# Autodesk Inventor assembly: main room, doors, corridor connected
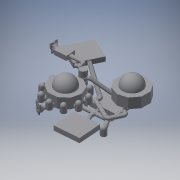
[picture p0: Inventor's stored thumbnail of the model, 180x180]
Saved by Autodesk Inventor 2017 (Build 210142000, 142)
## iProperties
Created: 2018-03-04
Part Number: main room, doors, corridor connected
Document SubType Name: Assembly
Designer: Braxton
Author: Braxton
## Documents named in this file (21)
- E:\School\Game develpment\geoscape\done solid\map\main room, doors, corridor connected.iam
- E:\School\Game develpment\geoscape\done solid\rooms\assembly\main room with double door.iam
- E:\School\Game develpment\geoscape\done solid\corridors\corridor.ipt
- E:\School\Game develpment\geoscape\done solid\corridors\corridor turn.ipt
- E:\School\Game develpment\geoscape\done solid\corridors\Y corridor.ipt
- E:\School\Game develpment\geoscape\done solid\corridors\end cap.ipt
- E:\School\Game develpment\geoscape\done solid\corridors\ramp top connect.ipt
- E:\School\Game develpment\geoscape\done solid\corridors\ramp.ipt
- E:\School\Game develpment\geoscape\done solid\corridors\ramp bottom connect.ipt
- E:\School\Game develpment\geoscape\done solid\corridors\curve ramp.ipt
- E:\School\Game develpment\geoscape\done solid\rooms\assembly\dome with double door.iam
- E:\School\Game develpment\geoscape\done solid\corridors\X corridor.ipt
- E:\School\Game develpment\geoscape\done solid\rooms\room with 15 cubicals.ipt
- E:\School\Game develpment\geoscape\done solid\corridors\ramp connect both ends.ipt
- E:\School\Game develpment\geoscape\done solid\doors\end door\9 foot door\end door room (9).ipt
- E:\School\Game develpment\geoscape\done solid\doors\end door\9 foot door\end door assembly (9).ipt.iam
- E:\School\Game develpment\geoscape\done solid\rooms\assembly\dome one terminal.iam
- E:\School\Game develpment\geoscape\done solid\rooms\assembly\assembly of dome with corridors with all doors.iam
- E:\School\Game develpment\geoscape\doors\end door assembly (closed) (9).ipt.iam
- end door assembly (9).ipt
- end door assembly (closed) (9).ipt
## Components (69 placed, 19 different names)
1. ramp top connect:3 — Flush:84, Insert:77, Flush:103, Insert:87
2. ramp:8 — Insert:74, Flush:81, Insert:75, Flush:82
3. ramp:7 — Insert:75, Flush:82, Insert:76, Flush:83
4. ramp:6 — Insert:73, Flush:80, Flush:84, Insert:77
5. ramp:5 — Insert:72, Flush:79, Insert:73, Flush:80
6. ramp:4 — Insert:72, Flush:79, Insert:74, Flush:81
7. ramp bottom connect:3 — Insert:71, Flush:78, Insert:76, Flush:83
8. corridor turn:8 — Insert:70, Flush:77, Insert:71, Flush:78
9. corridor turn:7 — Flush:75, Insert:68, Insert:70, Flush:77
10. corridor:18 — Flush:71, Insert:64, Flush:75, Insert:68
11. corridor:17 — Insert:65, Flush:72, Insert:66, Flush:73
12. corridor:16 — Insert:66, Flush:73, Flush:74, Insert:67
13. corridor:15 — Flush:71, Insert:64, Insert:65, Flush:72
14. corridor turn:6 — Flush:70, Insert:63, Flush:74, Insert:67
15. corridor:14 — Flush:68, Insert:61, Flush:70, Insert:63
16. corridor:13 — Flush:68, Insert:61, Insert:62, Flush:69
17. ramp top connect:2 — Flush:65, Insert:58, Flush:66, Insert:60
18. corridor turn:5 — Flush:67, Insert:59, Insert:62, Flush:69
19. corridor turn:4 — Flush:66, Flush:67, Insert:59, Insert:60
20. ramp bottom connect:2 — Flush:64, Insert:57, Flush:65, Insert:58
21. corridor:12 — Flush:56, Insert:50, Insert:51, Flush:60
22. corridor:11 — Insert:52, Insert:53, Flush:57, Flush:58
23. corridor:10 — Insert:53, Flush:57, Flush:59, Flush:61, Insert:55
24. ramp connect both ends:2 — Flush:46, Insert:45, Flush:48, Insert:47
25. ramp connect both ends:1 — Flush:47, Insert:46, Flush:49, Insert:48
26. Y corridor:2 — Insert:51, Insert:52, Flush:58, Flush:60, Flush:64, Insert:57
27. X corridor:1 — Flush:44, Insert:43, Flush:46, Flush:47, Insert:45, Insert:46, Flush:56, Insert:50
28. corridor:9 — Flush:43, Flush:44, Insert:42, Insert:43
29. corridor:8 — Flush:42, Flush:43, Insert:41, Insert:42
30. corridor turn:3 — Insert:40, Flush:41, Flush:42, Insert:41
31. curve ramp:1 — Flush:23, Insert:24, Flush:24, Insert:25, Flush:33, Insert:27, Flush:35, Insert:36, Flush:38, Insert:37, Insert:40, Flush:41, Flush:76, Insert:69
32. ramp top connect:1 — Flush:24, Insert:25, Flush:25, Insert:26
33. corridor turn:2 — Flush:28, Flush:33, Insert:27, Insert:28
34. corridor:3 — Flush:28, Flush:29, Insert:32, Flush:54, Insert:49
35. corridor:4 — Flush:29, Flush:30, Insert:31, Insert:32
36. corridor:5 — Flush:30, Flush:31, Insert:30, Insert:31
37. corridor:6 — Flush:31, Flush:32, Insert:29, Insert:30
38. corridor:7 — Flush:32, Insert:28, Insert:29
39. end cap:4 — Flush:35, Insert:36
40. end cap:5 — Flush:38, Insert:37
41. ramp bottom connect:1 — Flush:19, Insert:18, Flush:40, Insert:39
42. ramp:1 — Flush:17, Insert:20, Flush:25, Insert:26
43. ramp:2 — Flush:17, Flush:18, Insert:19, Insert:20
44. ramp:3 — Flush:18, Flush:19, Insert:18, Insert:19
45. corridor:1 — Flush:1, Flush:2, Insert:1, Insert:2
46. corridor:2 — Flush:2, Flush:3, Insert:2, Insert:3
47. corridor turn:1 — Flush:3, Flush:4, Insert:3, Insert:4
48. Y corridor:1 — Flush:4, Insert:4, Flush:23, Insert:24, Flush:104, Insert:88
49. end cap:1 — Flush:104, Insert:88
50. room with 15 cubicals:1 — Flush:48, Insert:47
51. room with 15 cubicals:2 — Flush:49, Insert:48
52. room with 15 cubicals:3 — Flush:103, Insert:87
53. dome one terminal:10 [sub-assembly] — Insert:81, Flush:93
54. dome one terminal:9 [sub-assembly] — Insert:82, Flush:92
55. dome one terminal:8 [sub-assembly] — Insert:83, Flush:91
56. dome one terminal:7 [sub-assembly] — Insert:86, Flush:90
57. dome one terminal:6 [sub-assembly] — Insert:85, Flush:89
58. dome one terminal:5 [sub-assembly] — Insert:84, Flush:88
59. dome one terminal:4 [sub-assembly] — Insert:80, Flush:87
60. dome one terminal:3 [sub-assembly] — Insert:79, Flush:86
61. dome one terminal:2 [sub-assembly] — Insert:78, Flush:85
62. assembly of dome with corridors with all doors:1 [sub-assembly] — Flush:76, Insert:69, Insert:78, Insert:79, Insert:80, Insert:81, Insert:82, Insert:83, Insert:84, Insert:85, Insert:86, Flush:85, Flush:86, Flush:87, Flush:88, Flush:89, Flush:90, Flush:91, Flush:92, Flush:93
63. dome one terminal:1 [sub-assembly] — Flush:59, Flush:61, Insert:55
64. dome with double door:1 [sub-assembly] — Flush:40, Insert:39
65. main room with double door:1 [sub-assembly] — Flush:1, Insert:1, Flush:106, Insert:89
66. end door assembly (closed) (9).ipt:1 [sub-assembly] — Flush:107, Mate:53, Mate:54
67. end door room (9):1 — Flush:54, Insert:49, Flush:55, Mate:47, Mate:48, Mate:51, Mate:52
68. end door assembly (9).ipt:1 [sub-assembly] — Flush:55, Mate:47, Mate:48, Mate:51, Mate:52
69. end door room (Starting) (9):2 — Flush:106, Insert:89, Flush:107, Mate:53, Mate:54
## Relationships (141: Flush 69, Insert 66, Mate 6)
- Flush:1: corridor:1 ↔ main room with double door:1
- Flush:2: corridor:1 ↔ corridor:2
- Flush:3: corridor:2 ↔ corridor turn:1
- Flush:4: corridor turn:1 ↔ Y corridor:1
- Insert:1: corridor:1 ↔ main room with double door:1
- Insert:2: corridor:1 ↔ corridor:2
- Insert:3: corridor:2 ↔ corridor turn:1
- Insert:4: corridor turn:1 ↔ Y corridor:1
- Flush:17: ramp:1 ↔ ramp:2
- Flush:18: ramp:2 ↔ ramp:3
- Flush:19: ramp bottom connect:1 ↔ ramp:3
- Insert:18: ramp bottom connect:1 ↔ ramp:3
- Insert:19: ramp:2 ↔ ramp:3
- Insert:20: ramp:1 ↔ ramp:2
- Flush:23: curve ramp:1 ↔ Y corridor:1
- Insert:24: curve ramp:1 ↔ Y corridor:1
- Flush:24: curve ramp:1 ↔ ramp top connect:1
- Insert:25: curve ramp:1 ↔ ramp top connect:1
- Flush:25: ramp top connect:1 ↔ ramp:1
- Insert:26: ramp top connect:1 ↔ ramp:1
- Flush:28: corridor turn:2 ↔ corridor:3
- Flush:29: corridor:3 ↔ corridor:4
- Flush:30: corridor:4 ↔ corridor:5
- Flush:31: corridor:5 ↔ corridor:6
- Flush:32: corridor:6 ↔ corridor:7
- Flush:33: curve ramp:1 ↔ corridor turn:2
- Insert:27: curve ramp:1 ↔ corridor turn:2
- Insert:28: corridor turn:2 ↔ corridor:7
- Insert:29: corridor:6 ↔ corridor:7
- Insert:30: corridor:5 ↔ corridor:6
- Insert:31: corridor:4 ↔ corridor:5
- Insert:32: corridor:3 ↔ corridor:4
- Flush:35: curve ramp:1 ↔ end cap:4
- Insert:36: curve ramp:1 ↔ end cap:4
- Flush:38: curve ramp:1 ↔ end cap:5
- Insert:37: curve ramp:1 ↔ end cap:5
- Flush:40: ramp bottom connect:1 ↔ dome with double door:1
- Insert:39: ramp bottom connect:1 ↔ dome with double door:1
- Insert:40: corridor turn:3 ↔ curve ramp:1
- Flush:41: corridor turn:3 ↔ curve ramp:1
- Flush:42: corridor:8 ↔ corridor turn:3
- Flush:43: corridor:9 ↔ corridor:8
- Flush:44: X corridor:1 ↔ corridor:9
- Insert:41: corridor:8 ↔ corridor turn:3
- Insert:42: corridor:9 ↔ corridor:8
- Insert:43: X corridor:1 ↔ corridor:9
- Flush:46: ramp connect both ends:2 ↔ X corridor:1
- Flush:47: ramp connect both ends:1 ↔ X corridor:1
- Insert:45: ramp connect both ends:2 ↔ X corridor:1
- Insert:46: ramp connect both ends:1 ↔ X corridor:1
- Flush:48: ramp connect both ends:2 ↔ room with 15 cubicals:1
- Insert:47: ramp connect both ends:2 ↔ room with 15 cubicals:1
- Flush:49: ramp connect both ends:1 ↔ room with 15 cubicals:2
- Insert:48: ramp connect both ends:1 ↔ room with 15 cubicals:2
- Flush:54: corridor:3 ↔ end door room (9):1
- Insert:49: corridor:3 ↔ end door room (9):1
- Flush:55: end door room (9):1 ↔ end door assembly (9).ipt:1
- Mate:47: end door room (9):1 ↔ end door assembly (9).ipt:1
- Mate:48: end door room (9):1 ↔ end door assembly (9).ipt:1
- Flush:56: corridor:12 ↔ X corridor:1
- Insert:50: corridor:12 ↔ X corridor:1
- Insert:51: corridor:12 ↔ Y corridor:2
- Insert:52: corridor:11 ↔ Y corridor:2
- Insert:53: corridor:11 ↔ corridor:10
- Flush:57: corridor:11 ↔ corridor:10
- Flush:58: corridor:11 ↔ Y corridor:2
- Flush:59: corridor:10 ↔ dome one terminal:1
- Flush:60: corridor:12 ↔ Y corridor:2
- Flush:61: corridor:10 ↔ dome one terminal:1
- Insert:55: corridor:10 ↔ dome one terminal:1
- Flush:64: ramp bottom connect:2 ↔ Y corridor:2
- Insert:57: ramp bottom connect:2 ↔ Y corridor:2
- Flush:65: ramp top connect:2 ↔ ramp bottom connect:2
- Insert:58: ramp top connect:2 ↔ ramp bottom connect:2
- Flush:66: ramp top connect:2 ↔ corridor turn:4
- Flush:67: corridor turn:5 ↔ corridor turn:4
- Insert:59: corridor turn:5 ↔ corridor turn:4
- Insert:60: ramp top connect:2 ↔ corridor turn:4
- Flush:68: corridor:14 ↔ corridor:13
- Insert:61: corridor:14 ↔ corridor:13
- Insert:62: corridor:13 ↔ corridor turn:5
- Flush:69: corridor:13 ↔ corridor turn:5
- Flush:70: corridor turn:6 ↔ corridor:14
- Insert:63: corridor turn:6 ↔ corridor:14
- Flush:71: corridor:18 ↔ corridor:15
- Insert:64: corridor:18 ↔ corridor:15
- Insert:65: corridor:17 ↔ corridor:15
- Flush:72: corridor:17 ↔ corridor:15
- Insert:66: corridor:17 ↔ corridor:16
- Flush:73: corridor:17 ↔ corridor:16
- Flush:74: corridor:16 ↔ corridor turn:6
- Insert:67: corridor:16 ↔ corridor turn:6
- Mate:51: end door room (9):1 ↔ end door assembly (9).ipt:1
- Mate:52: end door room (9):1 ↔ end door assembly (9).ipt:1
- Flush:75: corridor turn:7 ↔ corridor:18
- Insert:68: corridor turn:7 ↔ corridor:18
- Flush:76: curve ramp:1 ↔ assembly of dome with corridors with all doors:1
- Insert:69: curve ramp:1 ↔ assembly of dome with corridors with all doors:1
- Insert:70: corridor turn:8 ↔ corridor turn:7
- Flush:77: corridor turn:8 ↔ corridor turn:7
- Insert:71: ramp bottom connect:3 ↔ corridor turn:8
- Flush:78: ramp bottom connect:3 ↔ corridor turn:8
- Insert:72: ramp:5 ↔ ramp:4
- Flush:79: ramp:5 ↔ ramp:4
- Insert:73: ramp:6 ↔ ramp:5
- Flush:80: ramp:6 ↔ ramp:5
- Insert:74: ramp:8 ↔ ramp:4
- Flush:81: ramp:8 ↔ ramp:4
- Insert:75: ramp:8 ↔ ramp:7
- Flush:82: ramp:8 ↔ ramp:7
- Insert:76: ramp:7 ↔ ramp bottom connect:3
- Flush:83: ramp:7 ↔ ramp bottom connect:3
- Flush:84: ramp top connect:3 ↔ ramp:6
- Insert:77: ramp top connect:3 ↔ ramp:6
- Insert:78: dome one terminal:2 ↔ assembly of dome with corridors with all doors:1
- Insert:79: dome one terminal:3 ↔ assembly of dome with corridors with all doors:1
- Insert:80: dome one terminal:4 ↔ assembly of dome with corridors with all doors:1
- Insert:81: dome one terminal:10 ↔ assembly of dome with corridors with all doors:1
- Insert:82: dome one terminal:9 ↔ assembly of dome with corridors with all doors:1
- Insert:83: dome one terminal:8 ↔ assembly of dome with corridors with all doors:1
- Insert:84: dome one terminal:5 ↔ assembly of dome with corridors with all doors:1
- Insert:85: dome one terminal:6 ↔ assembly of dome with corridors with all doors:1
- Insert:86: dome one terminal:7 ↔ assembly of dome with corridors with all doors:1
- Flush:85: dome one terminal:2 ↔ assembly of dome with corridors with all doors:1
- Flush:86: dome one terminal:3 ↔ assembly of dome with corridors with all doors:1
- Flush:87: dome one terminal:4 ↔ assembly of dome with corridors with all doors:1
- Flush:88: dome one terminal:5 ↔ assembly of dome with corridors with all doors:1
- Flush:89: dome one terminal:6 ↔ assembly of dome with corridors with all doors:1
- Flush:90: dome one terminal:7 ↔ assembly of dome with corridors with all doors:1
- Flush:91: dome one terminal:8 ↔ assembly of dome with corridors with all doors:1
- Flush:92: dome one terminal:9 ↔ assembly of dome with corridors with all doors:1
- Flush:93: dome one terminal:10 ↔ assembly of dome with corridors with all doors:1
- Flush:103: ramp top connect:3 ↔ room with 15 cubicals:3
- Insert:87: ramp top connect:3 ↔ room with 15 cubicals:3
- Flush:104: Y corridor:1 ↔ end cap:1
- Insert:88: Y corridor:1 ↔ end cap:1
- Flush:106: main room with double door:1 ↔ end door room (Starting) (9):2
- Insert:89: main room with double door:1 ↔ end door room (Starting) (9):2
- Flush:107: end door assembly (closed) (9).ipt:1 ↔ end door room (Starting) (9):2
- Mate:53: end door assembly (closed) (9).ipt:1 ↔ end door room (Starting) (9):2
- Mate:54: end door assembly (closed) (9).ipt:1 ↔ end door room (Starting) (9):2
